# Autodesk Inventor assembly: Cosa sin eje
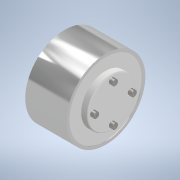
[picture p0: Inventor's stored thumbnail of the model, 180x180]
Saved by Autodesk Inventor 2021 (Build 250183000, 183)
## iProperties
Created: 2021-01-10
Part Number: Cosa sin eje
Document SubType Name: Assembly
Designer: dieku
Author: dieku
## Documents named in this file (7)
- C:\Users\dieku\Documents\GitHub\tallerDibujoIngenieria\Ensambles\Cosa sin eje.iam
- C:\Users\dieku\Documents\GitHub\tallerDibujoIngenieria\Ensambles\Rodamiento doble + arandela + cilindro separador.iam
- C:\Users\dieku\Documents\GitHub\tallerDibujoIngenieria\Partes\Cilindro Tensor.ipt
- C:\Users\dieku\Documents\GitHub\tallerDibujoIngenieria\Partes\Tapeta Exterior.ipt
- C:\Users\dieku\Documents\Inventor\Content Center Files\R2021\en-US\DIN 912\DIN 912 - M6 x 1 x 25 x 22,5.ipt
- C:\Users\dieku\Documents\GitHub\tallerDibujoIngenieria\Partes\tensorpolea.ipt
- C:\Users\dieku\Documents\GitHub\tallerDibujoIngenieria\Partes\Eje\Intento 1-1-2021\Ensamble 3 piezas final\DIN 912 - M6 x 1 x 16 x 13,5.ipt
## Components (12 placed, 6 different names)
1. Cilindro Tensor:1 — Insert:1, Insert:2, Insert:7, Insert:8
2. Rodamiento doble + arandela + cilindro separador:1 [sub-assembly] — Insert:1
3. Tapeta Exterior:1 — Insert:2, Insert:3, Insert:4, Insert:5, Insert:6
4. DIN 912 - replaced by DIN EN ISO 4762 M6 x 25:1 — Insert:3
5. DIN 912 - replaced by DIN EN ISO 4762 M6 x 25:2 — Insert:4
6. DIN 912 - replaced by DIN EN ISO 4762 M6 x 25:3 — Insert:5
7. DIN 912 - replaced by DIN EN ISO 4762 M6 x 25:4 — Insert:6
8. tensorpolea:1 — Insert:7, Insert:8, Insert:9, Insert:10, Insert:11, Insert:12
9. DIN 912 - M6 x 1 x 16 x 13,5:1 — Insert:10
10. DIN 912 - M6 x 1 x 16 x 13,5:2 — Insert:9
11. DIN 912 - M6 x 1 x 16 x 13,5:3 — Insert:11
12. DIN 912 - M6 x 1 x 16 x 13,5:4 — Insert:12
## Relationships (12: Insert 12)
- Insert:1: Cilindro Tensor:1 ↔ Rodamiento doble + arandela + cilindro separador:1
- Insert:2: Cilindro Tensor:1 ↔ Tapeta Exterior:1
- Insert:3: Tapeta Exterior:1 ↔ DIN 912 - replaced by DIN EN ISO 4762 M6 x 25:1
- Insert:4: Tapeta Exterior:1 ↔ DIN 912 - replaced by DIN EN ISO 4762 M6 x 25:2
- Insert:5: Tapeta Exterior:1 ↔ DIN 912 - replaced by DIN EN ISO 4762 M6 x 25:3
- Insert:6: Tapeta Exterior:1 ↔ DIN 912 - replaced by DIN EN ISO 4762 M6 x 25:4
- Insert:7: Cilindro Tensor:1 ↔ tensorpolea:1
- Insert:8: Cilindro Tensor:1 ↔ tensorpolea:1
- Insert:9 (-15 mm): tensorpolea:1 ↔ DIN 912 - M6 x 1 x 16 x 13,5:2
- Insert:10 (-15 mm): tensorpolea:1 ↔ DIN 912 - M6 x 1 x 16 x 13,5:1
- Insert:11 (-15 mm): tensorpolea:1 ↔ DIN 912 - M6 x 1 x 16 x 13,5:3
- Insert:12 (-15 mm): tensorpolea:1 ↔ DIN 912 - M6 x 1 x 16 x 13,5:4
